# Autodesk Inventor assembly: robot
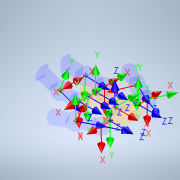
[picture p0: Inventor's stored thumbnail of the model, 180x180]
Saved by Autodesk Inventor 2020.2 (Build 242310000, 310)
## iProperties
Created: 2021-01-29
Part Number: robot
Document SubType Name: Assembly
Designer: DELL
Author: DELL
## Documents named in this file (7)
- D:\repo\FlexipodFast\mesh\v9.0\robot.iam
- D:\repo\FlexipodFast\mesh\v9.0\hip.ipt
- D:\repo\FlexipodFast\mesh\v9.0\thigh.ipt
- D:\repo\FlexipodFast\mesh\v9.0\shank_2.ipt
- D:\repo\FlexipodFast\mesh\v9.0\shank_front.ipt
- D:\repo\FlexipodFast\mesh\v9.0\body.ipt
- D:\repo\FlexipodFast\mesh\v9.0\shank_right.ipt
## Components (13 placed, 6 different names)
1. hip:1 — Rotational:1, Angle:34, Rotational:11
2. hip:2 — Rotational:2, Rotational:9, Angle:33
3. thigh:1 — Rotational:9, Rotational:15
4. thigh:2 — Rotational:10, Rotational:11
5. thigh:3 — Rotational:8, Rotational:21
6. thigh:4 — Rotational:12, Angle:36, Rotational:20
7. shank_2:3 — Angle:37, Rotational:20
8. shank_front:1 — Rotational:10
9. shank_front:2 — Rotational:15
10. hip:3 — Rotational:3, Rotational:8, Angle:35
11. hip:4 — Angle:29, Mate:64, Rotational:4, Rotational:12
12. body:1 — Flush:47, Flush:48, Flush:49, Angle:29, Mate:64, Rotational:1, Rotational:2, Rotational:3, Rotational:4, Angle:33, Angle:34, Angle:35, Angle:36, Angle:37
13. shank_right:1 — Rotational:21
## Relationships (22: RevoluteJoint 12, Angle 6, Flush 3, Mate 1)
- Flush:47: body:1
- Flush:48: body:1
- Flush:49: body:1
- Angle:29 (0 deg): hip:4 ↔ body:1
- Mate:64 (-71 mm): hip:4 ↔ body:1
- Rotational:1 [RevoluteJoint]: hip:1 ↔ body:1
- Rotational:2 [RevoluteJoint]: hip:2 ↔ body:1
- Rotational:3 [RevoluteJoint]: hip:3 ↔ body:1
- Rotational:4 [RevoluteJoint]: hip:4 ↔ body:1
- Rotational:8 [RevoluteJoint]: thigh:3 ↔ hip:3
- Rotational:9 [RevoluteJoint]: hip:2 ↔ thigh:1
- Angle:33 (0 deg): hip:2 ↔ body:1
- Angle:34 (180 deg): hip:1 ↔ body:1
- Angle:35 (180 deg): hip:3 ↔ body:1
- Rotational:10 [RevoluteJoint]: thigh:2 ↔ shank_front:1
- Rotational:11 [RevoluteJoint]: hip:1 ↔ thigh:2
- Rotational:12 [RevoluteJoint]: thigh:4 ↔ hip:4
- Rotational:15 [RevoluteJoint]: thigh:1 ↔ shank_front:2
- Angle:36 (0 deg): thigh:4 ↔ body:1
- Angle:37 (0 deg): shank_2:3 ↔ body:1
- Rotational:20 [RevoluteJoint]: thigh:4 ↔ shank_2:3
- Rotational:21 [RevoluteJoint]: thigh:3 ↔ shank_right:1
